# Autodesk Inventor assembly: MMCX_2DD-100P_Guide
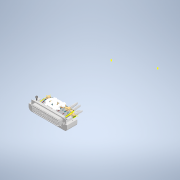
[picture p0: Inventor's stored thumbnail of the model, 180x180]
Saved by Autodesk Inventor 2020 (Build 240168000, 168)
## iProperties
Created: 2019-08-27
Part Number: MMCX_2DD-100P_Guide
Document SubType Name: Assembly
Designer: Eric
Author: Eric
## Documents named in this file (9)
- C:\Users\elmar\OneDrive\KiCAD\MMCX_2DD-100P\MMCX_2DD-100P_Guide.iam
- C:\Users\elmar\OneDrive\KiCAD\MMCX_2DD-100P\2DD-100P.ipt
- C:\Users\elmar\OneDrive\Inventor\Interlock\734151251.ipt
- C:\Users\elmar\OneDrive\KiCAD\MMCX_2DD-100P\PCtail.ipt
- C:\Users\elmar\OneDrive\KiCAD\MMCX_2DD-100P\MMCX_2DD-100P_Odd.iam
- C:\Users\elmar\OneDrive\KiCAD\MMCX_2DD-100P\MMCX_2DD-100P_Even.iam
- C:\Users\elmar\OneDrive\Documents\Inventor\Content Center Files\R2020\en-US\BS EN ISO 4762\BS EN ISO 4762 - M2 x 12(1).ipt
- C:\Users\elmar\OneDrive\KiCAD\MMCX_2DD-100P\HousingLogoPositive.ipt
- C:\Users\elmar\OneDrive\KiCAD\MMCX_2DD-100P\InsertionGuide.ipt
## Components (40 placed, 8 different names)
1. 2DD-100P:3 — Insert:1, Insert:2, Insert:3, Insert:4, Insert:5, Insert:6, Mate:3, Mate:4, Angle:5, Angle:6, Angle:7, Mate:5, Mate:7, Angle:8, Angle:9, Flush:2
2. 734151251:2 — Insert:7
3. 734151251:12 — Insert:10
4. 734151251:1 — Insert:9
5. 734151251:3 — Insert:8
6. MMCX_2DD-100P_Odd:1 [sub-assembly] — Angle:6, Angle:7, Mate:5, Mate:6, Insert:7, Insert:8, Flush:1, Tangent:3, Mate:8, Flush:3
7. MMCX_2DD-100P_Even:1 [sub-assembly] — Mate:7, Angle:8, Angle:9, Tangent:2, Flush:1, Insert:9, Insert:10, Flush:4
8. InsertionGuide:1 — Flush:2, Mate:8, Flush:3, Flush:4, Insert:11, Mate:9, Mate:10, Mate:11
9. BS EN ISO 4762 - Metric M2 x 12:1 — Insert:11
10. HousingLogoPositive:1 — Mate:9, Mate:10, Mate:11
11. PCtail:4 — Insert:3
12. PCtail:5 — Insert:1
13. PCtail:6 — Insert:6
14. PCtail:1 — Insert:2
15. PCtail:2 — Insert:4, Tangent:3
16. PCtail:3 — Insert:5
17. PCtail:7
18. PCtail:8
19. PCtail:9
20. PCtail:10
21. PCtail:11
22. PCtail:12
23. PCtail:13
24. PCtail:14
25. PCtail:15
26. PCtail:16
27. PCtail:17
28. PCtail:18
29. PCtail:19
30. PCtail:20
31. PCtail:21
32. PCtail:22 — Tangent:2
33. PCtail:23
34. PCtail:24
35. PCtail:25
36. PCtail:26
37. PCtail:27
38. PCtail:28
39. PCtail:29
40. PCtail:30
## Component patterns: (5 elements, first: PCtail:4 + PCtail:5 + PCtail:6 + PCtail:1 + PCtail:2 + PCtail:3)
## Relationships (31: Insert 11, Mate 9, Angle 5, Flush 4, Tangent 2)
- Insert:1: 2DD-100P:3 ↔ PCtail:5
- Insert:2: 2DD-100P:3 ↔ PCtail:1
- Insert:3: 2DD-100P:3 ↔ PCtail:4
- Insert:4: 2DD-100P:3 ↔ PCtail:2
- Insert:5: 2DD-100P:3 ↔ PCtail:3
- Insert:6: 2DD-100P:3 ↔ PCtail:6
- Mate:3: 2DD-100P:3
- Mate:4: 2DD-100P:3
- Angle:5 (0 deg): 2DD-100P:3
- Angle:6 (0 deg): 2DD-100P:3 ↔ MMCX_2DD-100P_Odd:1
- Angle:7 (-5 deg): 2DD-100P:3 ↔ MMCX_2DD-100P_Odd:1
- Mate:5: 2DD-100P:3 ↔ MMCX_2DD-100P_Odd:1
- Mate:6 (1.9517 mm): MMCX_2DD-100P_Odd:1
- Insert:7: 734151251:2 ↔ MMCX_2DD-100P_Odd:1
- Insert:8: 734151251:3 ↔ MMCX_2DD-100P_Odd:1
- Mate:7: 2DD-100P:3 ↔ MMCX_2DD-100P_Even:1
- Angle:8 (0 deg): 2DD-100P:3 ↔ MMCX_2DD-100P_Even:1
- Angle:9 (-5 deg): 2DD-100P:3 ↔ MMCX_2DD-100P_Even:1
- Tangent:2: MMCX_2DD-100P_Even:1 ↔ PCtail:22
- Flush:1 (-3.9034 mm): MMCX_2DD-100P_Odd:1 ↔ MMCX_2DD-100P_Even:1
- Insert:9: 734151251:1 ↔ MMCX_2DD-100P_Even:1
- Insert:10: 734151251:12 ↔ MMCX_2DD-100P_Even:1
- Tangent:3: MMCX_2DD-100P_Odd:1 ↔ PCtail:2
- Flush:2: 2DD-100P:3 ↔ InsertionGuide:1
- Mate:8: MMCX_2DD-100P_Odd:1 ↔ InsertionGuide:1
- Flush:3: MMCX_2DD-100P_Odd:1 ↔ InsertionGuide:1
- Flush:4: MMCX_2DD-100P_Even:1 ↔ InsertionGuide:1
- Insert:11: InsertionGuide:1 ↔ BS EN ISO 4762 - Metric M2 x 12:1
- Mate:9: InsertionGuide:1 ↔ HousingLogoPositive:1
- Mate:10: InsertionGuide:1 ↔ HousingLogoPositive:1
- Mate:11: InsertionGuide:1 ↔ HousingLogoPositive:1
## Named parameters: PinSpacing = 1.95171 mm, BoardAngle = -5 deg
